# Autodesk Inventor assembly: SubSistemaLiberacion
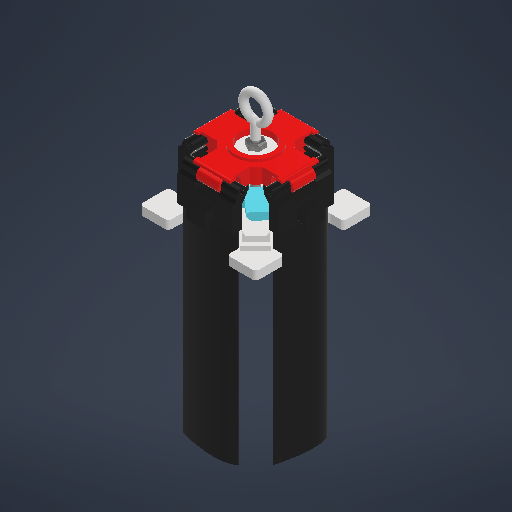
[picture p0: Inventor's stored thumbnail of the model, 512x512]
Saved by Autodesk Inventor 2026.1 (Build 301233000, 233)
## iProperties
Created: 2025-12-08
Part Number: SubSistemaLiberacion
Document SubType Name: Assembly
Designer: vickh
Author: vickh
## Documents named in this file (11)
- C:\Users\vickh\Documents\Proyectos\Cansat_Huitzilin\3D\NuevoDiseno\SubSistemaLiberacion.iam
- C:\Users\vickh\Documents\Proyectos\Cansat_Huitzilin\3D\NuevoDiseno\SujeccionHelices.ipt
- C:\Users\vickh\Documents\Proyectos\Cansat_Huitzilin\3D\NuevoDiseno\Pala.ipt
- C:\Users\vickh\Documents\Proyectos\Cansat_Huitzilin\3D\NuevoDiseno\SistemaLiberacion2.2.ipt
- C:\Users\vickh\Documents\Proyectos\Cansat_Huitzilin\3D\NuevoDiseno\SistemLiberacion1.ipt
- C:\Users\vickh\Downloads\628-ZZ-TheTimkenCompany-3D-01-17-2026\628-ZZ-TheTimkenCompany-3D-01-17-2026\628-ZZ-TheTimkenCompany-3D-01-17-2026.ipt
- C:\Users\vickh\Downloads\ArmellaCerrada.ipt
- C:\Users\vickh\Downloads\Tuerca1-4.ipt
- C:\Users\vickh\Downloads\ArandelaDeCaucho.ipt
- C:\Users\vickh\Downloads\Arandela1-4.ipt
- C:\Users\vickh\Downloads\SistemaDeDesacople.ipt
## Components (16 placed, 10 different names)
1. SujeccionHelices:1 — Coincidencia:9, De rotación:1, De rotación:2, De rotación:3, De rotación:4
2. Pala:1 — De rotación:3
3. Pala:2 — De rotación:2
4. Pala:3 — De rotación:4
5. Pala:4 — De rotación:1
6. SistemaLiberacion2.2:1
7. 628-ZZ-TheTimkenCompany-3D-01-17-2026:1 — Coincidencia:9, Insertar:5, Coincidencia:10
8. ArmellaCerrada:1 — Coincidencia:6, Insertar:6, Cilíndrica:1
9. Tuerca1-4:1 — Coincidencia:6, Coincidencia:7
10. ArandelaDeCaucho:1 — Coincidencia:8, Insertar:5
11. Arandela1-4:1 — Coincidencia:7, Coincidencia:8
12. ArandelaDeCaucho:2 — Coincidencia:10, Coincidencia:11
13. Arandela1-4:2 — Coincidencia:11, Coincidencia:12
14. Tuerca1-4:2 — Coincidencia:12
15. SistemaDeDesacople:1 — Insertar:6
16. SistemLiberacion1:1 — Cilíndrica:1
## Relationships (14: Mate 7, RevoluteJoint 4, Insert 2, CylindricalJoint 1)
- Coincidencia:6 [Mate]: ArmellaCerrada:1 ↔ Tuerca1-4:1
- Coincidencia:7 [Mate]: Tuerca1-4:1 ↔ Arandela1-4:1
- Coincidencia:8 [Mate]: ArandelaDeCaucho:1 ↔ Arandela1-4:1
- Coincidencia:9 [Mate]: SujeccionHelices:1 ↔ 628-ZZ-TheTimkenCompany-3D-01-17-2026:1
- Insertar:5: 628-ZZ-TheTimkenCompany-3D-01-17-2026:1 ↔ ArandelaDeCaucho:1
- Coincidencia:10 [Mate]: 628-ZZ-TheTimkenCompany-3D-01-17-2026:1 ↔ ArandelaDeCaucho:2
- Coincidencia:11 [Mate]: ArandelaDeCaucho:2 ↔ Arandela1-4:2
- Coincidencia:12 [Mate]: Arandela1-4:2 ↔ Tuerca1-4:2
- Insertar:6 (5 mm): ArmellaCerrada:1 ↔ SistemaDeDesacople:1
- De rotación:1 [RevoluteJoint]: SujeccionHelices:1 ↔ Pala:4
- De rotación:2 [RevoluteJoint]: SujeccionHelices:1 ↔ Pala:2
- De rotación:3 [RevoluteJoint]: SujeccionHelices:1 ↔ Pala:1
- De rotación:4 [RevoluteJoint]: SujeccionHelices:1 ↔ Pala:3
- Cilíndrica:1 [CylindricalJoint]: ArmellaCerrada:1 ↔ SistemLiberacion1:1
